# Autodesk Inventor assembly: BL6
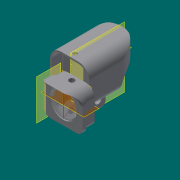
[picture p0: Inventor's stored thumbnail of the model, 180x180]
Saved by Autodesk Inventor 2016 (Build 200138000, 138)
## iProperties
Created: 2016-12-21
Part Number: BL6
Document SubType Name: Assembly
Designer: Student
Author: Student
## Documents named in this file (6)
- C:\Users\katzchristy\.babun\cygwin\home\katzchristy\samsbikelights\Bike_Light_Slide60\BL6.iam
- C:\Users\katzchristy\.babun\cygwin\home\katzchristy\samsbikelights\Lib_Light_Parts\Light PCB-complete.iam
- C:\Users\katzchristy\.babun\cygwin\home\katzchristy\samsbikelights\Bike_Light_Slide60\Rear.ipt
- C:\Users\katzchristy\.babun\cygwin\home\katzchristy\samsbikelights\Lib_Light_Parts\light LED.ipt
- C:\Users\katzchristy\.babun\cygwin\home\katzchristy\samsbikelights\Bike_Light_Slide60\Front.ipt
- C:\Users\katzchristy\.babun\cygwin\home\katzchristy\samsbikelights\Lib_Light_Parts\light Lens.ipt
## Components (5 placed, 5 different names)
1. Light PCB-complete:1 [sub-assembly] — Rigid:1
2. Rear:1
3. light LED:1 — Rigid:1
4. Front:1 — Rigid:2
5. light Lens:1 — Rigid:2
## Relationships (2: WeldJoint 2)
- Rigid:1 [WeldJoint] (1.524 mm): Light PCB-complete:1 ↔ light LED:1
- Rigid:2 [WeldJoint]: Front:1 ↔ light Lens:1
